# Autodesk Inventor assembly: Omni Assembly
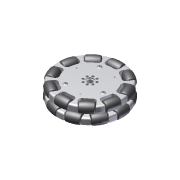
[picture p0: Inventor's stored thumbnail of the model, 180x180]
Saved by Autodesk Inventor 2015 (Build 190159000, 159)
## iProperties
Created: 2015-01-22
Part Number: Omni Assembly
Document SubType Name: Assembly
Designer: rihoobler
Author: rihoobler
## Documents named in this file (3)
- C:\Users\rihoobler\Documents\Inventor\SerenityMk.2\Omni Assembly.iam
- C:\Users\rihoobler\Documents\Inventor\SerenityMk.2\Imported Components\tetrix_736466_2012\tetrix_736466_2012.iam
- C:\Users\rihoobler\Documents\Inventor\SerenityMk.2\Imported Components\tetrix_739172_2012\tetrix_739172_2012.iam
## Components (3 placed, 2 different names)
1. tetrix_736466_2012:1 [sub-assembly] — Insert:1
2. tetrix_736466_2012:2 [sub-assembly] — Mate:1, Mate:2
3. tetrix_739172_2012:1 [sub-assembly] — Insert:1, Mate:1, Mate:2
## Relationships (3: Mate 2, Insert 1)
- Insert:1: tetrix_736466_2012:1 ↔ tetrix_739172_2012:1
- Mate:1: tetrix_736466_2012:2 ↔ tetrix_739172_2012:1
- Mate:2: tetrix_736466_2012:2 ↔ tetrix_739172_2012:1
